# Autodesk Inventor assembly: Schlitten
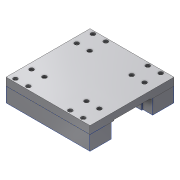
[picture p0: Inventor's stored thumbnail of the model, 180x180]
Saved by Autodesk Inventor 2016 (Build 200138000, 138)
## iProperties
Created: 2015-08-05
Part Number: Schlitten
Document SubType Name: Assembly
## Documents named in this file (3)
- E:\GitHub\CNC-Router_Z-Axis\Schlitten.iam
- E:\GitHub\CNC-Router_Z-Axis\Befestigungsplatte.ipt
- E:\GitHub\CNC-Router_Z-Axis\Distanzblock.ipt
## Components (3 placed, 2 different names)
1. Befestigungsplatte:1 — Flush:5, Flush:6, Flush:7, Mate:1, Mate:2
2. Distanzblock:1 — Mate:2
3. Distanzblock:2 — Mate:1
## Relationships (9: Flush 7, Mate 2)
- [Flush]: Befestigungsplatte:1 ↔ Distanzblock:2
- [Flush]: Befestigungsplatte:1 ↔ Distanzblock:2
- [Flush]: Befestigungsplatte:1 ↔ Distanzblock:1
- [Flush]: Befestigungsplatte:1 ↔ Distanzblock:1
- Flush:5: Befestigungsplatte:1
- Flush:6: Befestigungsplatte:1
- Flush:7: Befestigungsplatte:1
- Mate:1: Befestigungsplatte:1 ↔ Distanzblock:2
- Mate:2: Befestigungsplatte:1 ↔ Distanzblock:1
